# Autodesk Inventor assembly: 05-22-2023 assieme flangia-verga-curva
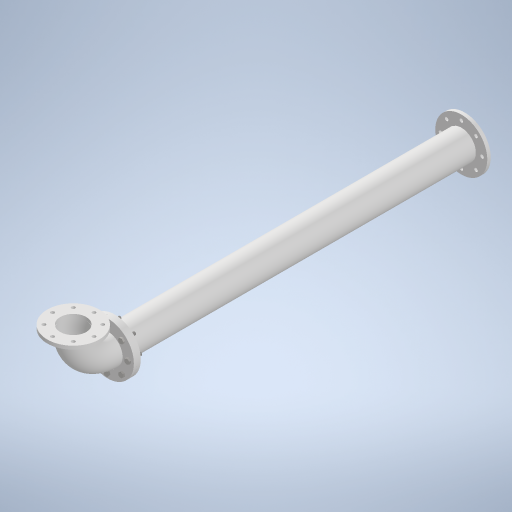
[picture p0: Inventor's stored thumbnail of the model, 512x512]
Saved by Autodesk Inventor 2023 (Build 270158000, 158)
## iProperties
Created: 2023-05-22
Part Number: 05-22-2023 assieme flangia-verga-curva
Document SubType Name: Assembly
Designer: Admin
Author: Admin
## Documents named in this file (7)
- C:\Users\Admin\Desktop\3DDDD\05-22-2023 assieme flangia-verga-curva.iam
- C:\Users\Admin\Desktop\3DDDD\05-22-2023 flangia.ipt
- C:\Users\Admin\Desktop\3DDDD\05-22-2023 verga.ipt
- C:\Users\Admin\Desktop\3DDDD\05-22-2023 curva Sweep.ipt
- C:\Users\Admin\Documents\Inventor\Content Center Files\R2023\it-IT\BS EN ISO 4017\BS EN ISO 4017 - M18 x 70BS EN.ipt
- C:\Users\Admin\Documents\Inventor\Content Center Files\R2023\it-IT\AS 1112 (4)\AS 1112 - M18(2).ipt
- C:\Users\Admin\Documents\Inventor\Content Center Files\R2023\it-IT\AS 1237 (3.1)\AS 1237 - 18 mm(1)Aluminium-6061.ipt
## Components (30 placed, 6 different names)
1. 05-22-2023 flangia:1 — Coincidente:1, Coincidente:2, Coincidente:3, Coincidente:6
2. 05-22-2023 verga:1 — Coincidente:1, Coincidente:2, Coincidente:3, Coincidente:4, Coincidente:5, Allineato:1
3. 05-22-2023 flangia:2 — Coincidente:4, Coincidente:5, Coincidente:6, Coincidente:11, Coincidente:12, Coincidente:13, Coincidente:20
4. 05-22-2023 curva Sweep:1 — Coincidente:7, Coincidente:8, Coincidente:9, Coincidente:10, Allineato:1
5. 05-22-2023 flangia:3 — Coincidente:7, Coincidente:8, Coincidente:11, Coincidente:12, Coincidente:13, Coincidente:14, Coincidente:15, Coincidente:16
6. 05-22-2023 flangia:4 — Coincidente:9, Coincidente:10, Coincidente:14
7. BS EN ISO 4017 - Metrico M18 x 70:1 — Coincidente:15, Coincidente:16, Coincidente:17, Coincidente:19
8. AS 1112 (4) - Metrico M18:1 — Coincidente:17, Coincidente:21
9. AS 1237 (3.1) 18 mm - Alluminio 6061:1 — Coincidente:19, Coincidente:20, Coincidente:21
10. BS EN ISO 4017 - Metrico M18 x 70:2
11. AS 1112 (4) - Metrico M18:2
12. AS 1237 (3.1) 18 mm - Alluminio 6061:2
13. BS EN ISO 4017 - Metrico M18 x 70:3
14. AS 1112 (4) - Metrico M18:3
15. AS 1237 (3.1) 18 mm - Alluminio 6061:3
16. BS EN ISO 4017 - Metrico M18 x 70:4
17. AS 1112 (4) - Metrico M18:4
18. AS 1237 (3.1) 18 mm - Alluminio 6061:4
19. BS EN ISO 4017 - Metrico M18 x 70:5
20. AS 1112 (4) - Metrico M18:5
21. AS 1237 (3.1) 18 mm - Alluminio 6061:5
22. BS EN ISO 4017 - Metrico M18 x 70:6
23. AS 1112 (4) - Metrico M18:6
24. AS 1237 (3.1) 18 mm - Alluminio 6061:6
25. BS EN ISO 4017 - Metrico M18 x 70:7
26. AS 1112 (4) - Metrico M18:7
27. AS 1237 (3.1) 18 mm - Alluminio 6061:7
28. BS EN ISO 4017 - Metrico M18 x 70:8
29. AS 1112 (4) - Metrico M18:8
30. AS 1237 (3.1) 18 mm - Alluminio 6061:8
## Component patterns: (8 elements, first: BS EN ISO 4017 - Metrico M18 x 70:1 + AS 1112 (4) - Metrico M18:1 + AS 1237 (3.1) 18 mm - Alluminio 6061:1)
## Relationships (21: Mate 20, Flush 1)
- Coincidente:1 [Mate]: 05-22-2023 flangia:1 ↔ 05-22-2023 verga:1
- Coincidente:2 [Mate]: 05-22-2023 flangia:1 ↔ 05-22-2023 verga:1
- Coincidente:3 [Mate]: 05-22-2023 flangia:1 ↔ 05-22-2023 verga:1
- Coincidente:4 [Mate]: 05-22-2023 verga:1 ↔ 05-22-2023 flangia:2
- Coincidente:5 [Mate]: 05-22-2023 verga:1 ↔ 05-22-2023 flangia:2
- Coincidente:6 [Mate]: 05-22-2023 flangia:1 ↔ 05-22-2023 flangia:2
- Coincidente:7 [Mate]: 05-22-2023 curva Sweep:1 ↔ 05-22-2023 flangia:3
- Coincidente:8 [Mate]: 05-22-2023 curva Sweep:1 ↔ 05-22-2023 flangia:3
- Coincidente:9 [Mate]: 05-22-2023 curva Sweep:1 ↔ 05-22-2023 flangia:4
- Coincidente:10 [Mate]: 05-22-2023 curva Sweep:1 ↔ 05-22-2023 flangia:4
- Coincidente:11 [Mate]: 05-22-2023 flangia:2 ↔ 05-22-2023 flangia:3
- Coincidente:12 [Mate]: 05-22-2023 flangia:2 ↔ 05-22-2023 flangia:3
- Coincidente:13 [Mate]: 05-22-2023 flangia:2 ↔ 05-22-2023 flangia:3
- Allineato:1 [Flush]: 05-22-2023 verga:1 ↔ 05-22-2023 curva Sweep:1
- Coincidente:14 [Mate]: 05-22-2023 flangia:3 ↔ 05-22-2023 flangia:4
- Coincidente:15 [Mate]: 05-22-2023 flangia:3 ↔ BS EN ISO 4017 - Metrico M18 x 70:1
- Coincidente:16 [Mate]: 05-22-2023 flangia:3 ↔ BS EN ISO 4017 - Metrico M18 x 70:1
- Coincidente:17 [Mate]: BS EN ISO 4017 - Metrico M18 x 70:1 ↔ AS 1112 (4) - Metrico M18:1
- Coincidente:19 [Mate]: BS EN ISO 4017 - Metrico M18 x 70:1 ↔ AS 1237 (3.1) 18 mm - Alluminio 6061:1
- Coincidente:20 [Mate]: 05-22-2023 flangia:2 ↔ AS 1237 (3.1) 18 mm - Alluminio 6061:1
- Coincidente:21 [Mate]: AS 1112 (4) - Metrico M18:1 ↔ AS 1237 (3.1) 18 mm - Alluminio 6061:1
